# Autodesk Inventor assembly: 1010_with_tnut
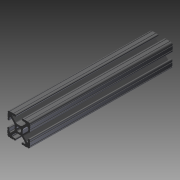
[picture p0: Inventor's stored thumbnail of the model, 180x180]
Saved by Autodesk Inventor 2015 (Build 190159000, 159)
## iProperties
Created: 2017-04-21
Part Number: 1010_with_tnut
Document SubType Name: Assembly
Designer: Raghava
Author: Raghava
## Documents named in this file (3)
- C:\Users\Raghava\Desktop\jackal_model\8020 Components\1010_with_tnut.iam
- C:\Users\Raghava\Desktop\jackal_model\8020 Components\1010_160mm.ipt
- C:\Users\Raghava\Desktop\jackal_model\8020 Components\14162_m.ipt
## Components (3 placed, 2 different names)
1. 1010_160mm:1 — Mate:1, Mate:2, Mate:3, Mate:4, Mate:5, Mate:6
2. 14162_m:1 — Mate:2, Mate:4, Mate:6, Mate:8
3. 14162_m:2 — Mate:1, Mate:3, Mate:5, Mate:7
## Relationships (9: Mate 9)
- Mate:1: 1010_160mm:1 ↔ 14162_m:2
- Mate:2: 1010_160mm:1 ↔ 14162_m:1
- Mate:3 (1.524 mm): 1010_160mm:1 ↔ 14162_m:2
- Mate:4 (1.524 mm): 1010_160mm:1 ↔ 14162_m:1
- Mate:5: 1010_160mm:1 ↔ 14162_m:2
- Mate:6: 1010_160mm:1 ↔ 14162_m:1
- Mate:7: 14162_m:2
- Mate:8: 14162_m:1
- Mate:9 (120 mm)
